# Autodesk Inventor assembly: FuseBlock
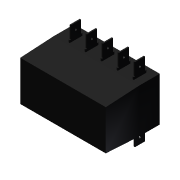
[picture p0: Inventor's stored thumbnail of the model, 180x180]
Saved by Autodesk Inventor 2015 (Build 190159000, 159)
## iProperties
Created: 2014-08-03
Part Number: FuseBlock
Document SubType Name: Assembly
Designer: david
Author: david
## Documents named in this file (2)
- C:\SharedDrive\Dropbox\FAST Robotics\Products\FAST_ROVER\810002_ASY-FAST ROVER v2\813006_FAST ROVER v2 CHASSIS ELECTRONICS\FuseBlock.iam
- C:\SharedDrive\Dropbox\FAST Robotics\Products\FAST_ROVER\810002_ASY-FAST ROVER v2\813006_FAST ROVER v2 CHASSIS ELECTRONICS\FuseBlock.ipt
## Components (1 placed, 1 different names)
1. FuseBlock:1 — Mate:1, Flush:1, Flush:2
## Relationships (3: Flush 2, Mate 1)
- Mate:1: FuseBlock:1
- Flush:1: FuseBlock:1
- Flush:2: FuseBlock:1
